# Autodesk Inventor assembly: BMS
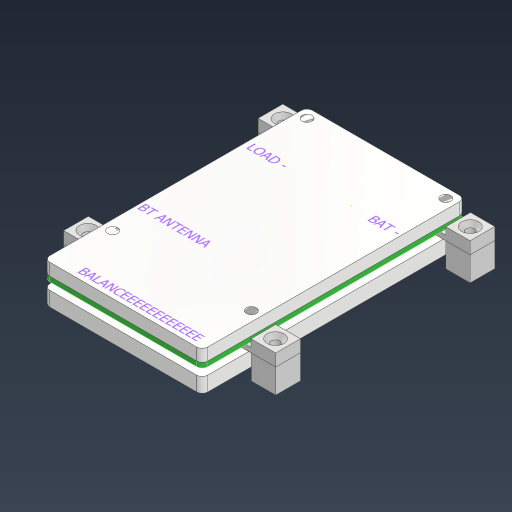
[picture p0: Inventor's stored thumbnail of the model, 512x512]
Saved by Autodesk Inventor 2023 (Build 270158000, 158)
## iProperties
Created: 2026-01-23
Part Number: BMS
Document SubType Name: Assembly
Designer: szymo
Author: szymo
## Documents named in this file (4)
- D:\tech\diy\e-skateboard\projekcik-inventor\BMS.iam
- D:\tech\diy\e-skateboard\projekcik-inventor\LLT 12S Li-ion 20A BMS v1.iam
- D:\tech\diy\e-skateboard\projekcik-inventor\BMS_hold_check.ipt
- D:\tech\diy\e-skateboard\projekcik-inventor\bms_hold_2.ipt
## Components (3 placed, 3 different names)
1. BMS_hold_check:1
2. bms_hold_2:1
3. LLT 12S Li-ion 20A BMS v1:1 [sub-assembly]
## Relationships (3: Flush 3)
- [Flush]: BMS_hold_check:1 ↔ LLT 12S Li-ion 20A BMS v1:1
- [Flush]: BMS_hold_check:1 ↔ LLT 12S Li-ion 20A BMS v1:1
- [Flush]: BMS_hold_check:1 ↔ bms_hold_2:1
